# Autodesk Inventor assembly: helatsm
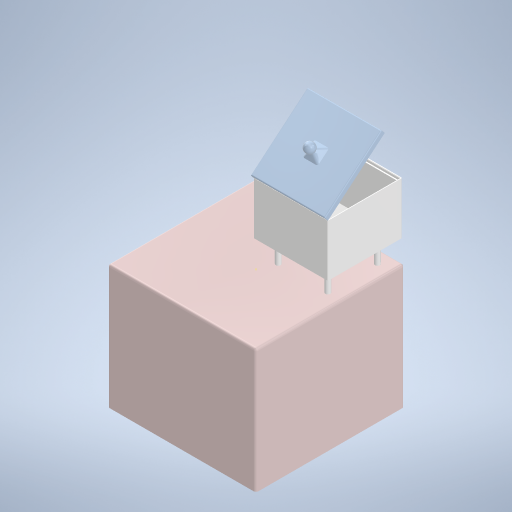
[picture p0: Inventor's stored thumbnail of the model, 512x512]
Saved by Autodesk Inventor 2023 (Build 270158000, 158)
## iProperties
Created: 2022-11-26
Part Number: helatsm
Document SubType Name: Assembly
Designer: abdul
Author: abdul
## Documents named in this file (5)
- C:\Users\abdul\OneDrive\Skrivbord\maskin design\cad\helatsm.iam
- C:\Users\abdul\OneDrive\Skrivbord\maskin design\cad\case.ipt
- C:\Users\abdul\OneDrive\Skrivbord\maskin design\cad\coffe container.ipt
- C:\Users\abdul\OneDrive\Skrivbord\maskin design\cad\coffee container lock.ipt
- C:\Users\abdul\OneDrive\Skrivbord\maskin design\cad\malare.ipt
## Components (5 placed, 4 different names)
1. case:1 — Mate:1, Mate:2, Mate:3, Mate:4, Mate:5, Flush:3, Flush:4, Flush:5, Mate:7, Mate:8
2. coffe container:1 — Mate:1, Mate:2, Mate:3, Mate:4, Mate:5, Mate:6, Flush:1
3. coffee container lock:1 — Mate:6, Flush:1
4. malare:1 — Flush:2, Flush:3, Flush:5, Mate:7
5. malare:2 — Flush:2, Flush:4, Mate:8
## Relationships (13: Mate 8, Flush 5)
- Mate:1: case:1 ↔ coffe container:1
- Mate:2: case:1 ↔ coffe container:1
- Mate:3: case:1 ↔ coffe container:1
- Mate:4: case:1 ↔ coffe container:1
- Mate:5: case:1 ↔ coffe container:1
- Mate:6: coffe container:1 ↔ coffee container lock:1
- Flush:1: coffe container:1 ↔ coffee container lock:1
- Flush:2: malare:1 ↔ malare:2
- Flush:3: case:1 ↔ malare:1
- Flush:4: case:1 ↔ malare:2
- Flush:5: case:1 ↔ malare:1
- Mate:7: case:1 ↔ malare:1
- Mate:8: case:1 ↔ malare:2
